# Autodesk Inventor assembly: Ensamble_chasis
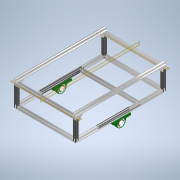
[picture p0: Inventor's stored thumbnail of the model, 180x180]
Saved by Autodesk Inventor 2022 (Build 260153000, 153)
## iProperties
Created: 2020-11-04
Part Number: Ensamble_chasis
Document SubType Name: Assembly
Designer: Cerberus 1S
Author: Cerberus 1S
## Documents named in this file (10)
- C:\Users\juanp\Desktop\Robocol\EVA\Recursos\Chasis\Diseño 1.3 (2020)\Ensamble_chasis.iam
- C:\Users\juanp\Desktop\Robocol\EVA\Recursos\Chasis\Diseño 1.3 (2020)\3 side holder.ipt
- C:\Users\juanp\Desktop\Robocol\EVA\Recursos\Chasis\Diseño 1.3 (2020)\20x20mm E.ipt
- C:\Users\juanp\Desktop\Robocol\EVA\Recursos\Chasis\Diseño 1.3 (2020)\20x20mm F.ipt
- C:\Users\juanp\Desktop\Robocol\EVA\Recursos\Chasis\Diseño 1.3 (2020)\20x20mm L_S.ipt
- C:\Users\juanp\Desktop\Robocol\EVA\Recursos\Chasis\Diseño 1.3 (2020)\20x20mm F_S.ipt
- C:\Users\juanp\Desktop\Robocol\EVA\Recursos\Chasis\Diseño 1.3 (2020)\20x20mm L.ipt
- C:\Users\juanp\Desktop\Robocol\EVA\Recursos\Chasis\Diseño 1.3 (2020)\Angulo S.ipt
- C:\Users\juanp\Desktop\Robocol\EVA\Recursos\Chasis\Diseño 1.3 (2020)\Pasador.ipt
- C:\Users\juanp\Desktop\Robocol\EVA\Recursos\Chasis\Diseño 1.3 (2020)\Soporte_chumacera.iam
## Components (25 placed, 9 different names)
1. 20x20mm E:1 — Coincidencia:1, Nivelación:1, Nivelación:2, Coincidencia:2, Nivelación:3, Nivelación:35, Coincidencia:19
2. 20x20mm E:2 — Nivelación:9, Coincidencia:4, Coincidencia:5, Nivelación:10, Coincidencia:14, Nivelación:24, Nivelación:25, Nivelación:64
3. 20x20mm E:3 — Coincidencia:9, Nivelación:18, Coincidencia:11, Nivelación:22, Nivelación:23, Coincidencia:13, Nivelación:33, Nivelación:34, Coincidencia:20, Nivelación:38
4. 20x20mm E:4 — Nivelación:20, Nivelación:21, Coincidencia:12, Coincidencia:18, Nivelación:32
5. 20x20mm F:1 — Coincidencia:2, Nivelación:3, Nivelación:4, Nivelación:7, Nivelación:8, Nivelación:9, Coincidencia:5, Nivelación:36, Coincidencia:71
6. 20x20mm F:2 — Nivelación:17, Nivelación:18, Coincidencia:11, Nivelación:19, Coincidencia:18
7. 3 side holder:1 — Nivelación:19, Nivelación:20, Nivelación:21, Coincidencia:12
8. 3 side holder:2 — Coincidencia:1, Nivelación:1, Nivelación:2, Nivelación:4
9. 3 side holder:3 — Nivelación:7, Nivelación:8, Coincidencia:4, Nivelación:10
10. 3 side holder:4 — Coincidencia:9, Nivelación:17, Nivelación:33, Nivelación:34, Nivelación:37
11. 20x20mm F_S:1 — Coincidencia:14, Nivelación:24, Nivelación:25, Nivelación:26, Nivelación:27, Coincidencia:15, Nivelación:28, Nivelación:29, Coincidencia:16, Coincidencia:28, Coincidencia:60, Coincidencia:61, Coincidencia:62, Nivelación:65
12. 20x20mm F_S:2 — Nivelación:22, Nivelación:23, Coincidencia:13, Nivelación:30, Nivelación:31, Coincidencia:17, Nivelación:32, Coincidencia:26, Coincidencia:27
13. 20x20mm L_S:1 — Nivelación:26, Nivelación:27, Coincidencia:15, Nivelación:30, Nivelación:31, Coincidencia:17, Coincidencia:23, Nivelación:40, Coincidencia:59, Coincidencia:65, Nivelación:66, Coincidencia:66, Symmetry:1
14. 20x20mm L_S:2 — Nivelación:28, Nivelación:29, Coincidencia:16, Coincidencia:21, Coincidencia:22, Nivelación:41, Nivelación:42, Symmetry:1
15. 20x20mm L:1 — Nivelación:35, Nivelación:36, Coincidencia:19, Nivelación:67, Coincidencia:69, Nivelación:68, Nivelación:69
16. 20x20mm L:2 — Coincidencia:20, Nivelación:37, Nivelación:38, Nivelación:70, Nivelación:71
17. Angulo S:1 — Coincidencia:21, Coincidencia:28, Nivelación:41
18. Angulo S:3 — Coincidencia:22, Coincidencia:27, Nivelación:42
19. Angulo S:4 — Coincidencia:23, Coincidencia:26, Nivelación:40
20. Angulo S:5 — Nivelación:64, Coincidencia:59, Coincidencia:60
21. Pasador:1 — Coincidencia:61, Coincidencia:62, Nivelación:65
22. Pasador:2 — Coincidencia:65, Nivelación:66, Coincidencia:66
23. 20x20mm F:3 — Nivelación:67, Coincidencia:69
24. Soporte_chumacera:3 [sub-assembly] — Nivelación:70, Nivelación:71, Coincidencia:70, Coincidencia:71
25. Soporte_chumacera:4 [sub-assembly] — Nivelación:68, Nivelación:69, Coincidencia:70
## Relationships (72: Flush 41, Mate 30, Symmetry 1)
- Coincidencia:1 [Mate]: 20x20mm E:1 ↔ 3 side holder:2
- Nivelación:1 [Flush]: 20x20mm E:1 ↔ 3 side holder:2
- Nivelación:2 [Flush]: 20x20mm E:1 ↔ 3 side holder:2
- Coincidencia:2 [Mate]: 20x20mm E:1 ↔ 20x20mm F:1
- Nivelación:3 [Flush]: 20x20mm E:1 ↔ 20x20mm F:1
- Nivelación:4 [Flush]: 20x20mm F:1 ↔ 3 side holder:2
- Nivelación:7 [Flush]: 20x20mm F:1 ↔ 3 side holder:3
- Nivelación:8 [Flush]: 20x20mm F:1 ↔ 3 side holder:3
- Nivelación:9 [Flush]: 20x20mm E:2 ↔ 20x20mm F:1
- Coincidencia:4 [Mate]: 20x20mm E:2 ↔ 3 side holder:3
- Coincidencia:5 [Mate]: 20x20mm E:2 ↔ 20x20mm F:1
- Nivelación:10 [Flush]: 20x20mm E:2 ↔ 3 side holder:3
- Coincidencia:9 [Mate]: 20x20mm E:3 ↔ 3 side holder:4
- Nivelación:17 [Flush]: 20x20mm F:2 ↔ 3 side holder:4
- Nivelación:18 [Flush]: 20x20mm E:3 ↔ 20x20mm F:2
- Coincidencia:11 [Mate]: 20x20mm E:3 ↔ 20x20mm F:2
- Nivelación:19 [Flush]: 20x20mm F:2 ↔ 3 side holder:1
- Nivelación:20 [Flush]: 20x20mm E:4 ↔ 3 side holder:1
- Nivelación:21 [Flush]: 20x20mm E:4 ↔ 3 side holder:1
- Coincidencia:12 [Mate]: 20x20mm E:4 ↔ 3 side holder:1
- Nivelación:22 [Flush]: 20x20mm E:3 ↔ 20x20mm F_S:2
- Nivelación:23 [Flush]: 20x20mm E:3 ↔ 20x20mm F_S:2
- Coincidencia:13 [Mate]: 20x20mm E:3 ↔ 20x20mm F_S:2
- Coincidencia:14 [Mate]: 20x20mm E:2 ↔ 20x20mm F_S:1
- Nivelación:24 [Flush]: 20x20mm E:2 ↔ 20x20mm F_S:1
- Nivelación:25 [Flush]: 20x20mm E:2 ↔ 20x20mm F_S:1
- Nivelación:26 [Flush]: 20x20mm F_S:1 ↔ 20x20mm L_S:1
- Nivelación:27 [Flush]: 20x20mm F_S:1 ↔ 20x20mm L_S:1
- Coincidencia:15 [Mate]: 20x20mm F_S:1 ↔ 20x20mm L_S:1
- Nivelación:28 [Flush]: 20x20mm F_S:1 ↔ 20x20mm L_S:2
- Nivelación:29 [Flush]: 20x20mm F_S:1 ↔ 20x20mm L_S:2
- Coincidencia:16 [Mate]: 20x20mm F_S:1 ↔ 20x20mm L_S:2
- Nivelación:30 [Flush]: 20x20mm F_S:2 ↔ 20x20mm L_S:1
- Nivelación:31 [Flush]: 20x20mm F_S:2 ↔ 20x20mm L_S:1
- Coincidencia:17 [Mate]: 20x20mm F_S:2 ↔ 20x20mm L_S:1
- Coincidencia:18 [Mate]: 20x20mm E:4 ↔ 20x20mm F:2
- Nivelación:32 [Flush]: 20x20mm E:4 ↔ 20x20mm F_S:2
- Nivelación:33 [Flush]: 20x20mm E:3 ↔ 3 side holder:4
- Nivelación:34 [Flush]: 20x20mm E:3 ↔ 3 side holder:4
- Nivelación:35 [Flush]: 20x20mm E:1 ↔ 20x20mm L:1
- Nivelación:36 [Flush]: 20x20mm F:1 ↔ 20x20mm L:1
- Coincidencia:19 [Mate]: 20x20mm E:1 ↔ 20x20mm L:1
- Coincidencia:20 [Mate]: 20x20mm E:3 ↔ 20x20mm L:2
- Nivelación:37 [Flush]: 3 side holder:4 ↔ 20x20mm L:2
- Nivelación:38 [Flush]: 20x20mm E:3 ↔ 20x20mm L:2
- Coincidencia:21 [Mate]: 20x20mm L_S:2 ↔ Angulo S:1
- Coincidencia:22 [Mate]: 20x20mm L_S:2 ↔ Angulo S:3
- Coincidencia:23 [Mate]: 20x20mm L_S:1 ↔ Angulo S:4
- Coincidencia:26 [Mate]: 20x20mm F_S:2 ↔ Angulo S:4
- Coincidencia:27 [Mate]: 20x20mm F_S:2 ↔ Angulo S:3
- Coincidencia:28 [Mate]: 20x20mm F_S:1 ↔ Angulo S:1
- Nivelación:40 [Flush]: 20x20mm L_S:1 ↔ Angulo S:4
- Nivelación:41 [Flush]: 20x20mm L_S:2 ↔ Angulo S:1
- Nivelación:42 [Flush]: 20x20mm L_S:2 ↔ Angulo S:3
- Nivelación:64 [Flush]: 20x20mm E:2 ↔ Angulo S:5
- Coincidencia:59 [Mate]: 20x20mm L_S:1 ↔ Angulo S:5
- Coincidencia:60 [Mate]: 20x20mm F_S:1 ↔ Angulo S:5
- Coincidencia:61 [Mate]: 20x20mm F_S:1 ↔ Pasador:1
- Coincidencia:62 [Mate]: 20x20mm F_S:1 ↔ Pasador:1
- Nivelación:65 [Flush]: 20x20mm F_S:1 ↔ Pasador:1
- Coincidencia:65 [Mate]: 20x20mm L_S:1 ↔ Pasador:2
- Nivelación:66 [Flush] (25 mm): 20x20mm L_S:1 ↔ Pasador:2
- Coincidencia:66 [Mate]: 20x20mm L_S:1 ↔ Pasador:2
- Nivelación:67 [Flush]: 20x20mm L:1 ↔ 20x20mm F:3
- Coincidencia:69 [Mate]: 20x20mm L:1 ↔ 20x20mm F:3
- Nivelación:68 [Flush]: 20x20mm L:1 ↔ Soporte_chumacera:4
- Nivelación:69 [Flush]: 20x20mm L:1 ↔ Soporte_chumacera:4
- Nivelación:70 [Flush]: 20x20mm L:2 ↔ Soporte_chumacera:3
- Nivelación:71 [Flush]: 20x20mm L:2 ↔ Soporte_chumacera:3
- Coincidencia:70 [Mate]: Soporte_chumacera:3 ↔ Soporte_chumacera:4
- Coincidencia:71 [Mate] (-320 mm): 20x20mm F:1 ↔ Soporte_chumacera:3
- Symmetry:1: 20x20mm L_S:1 ↔ 20x20mm L_S:2
